# Autodesk Inventor assembly: Osnova
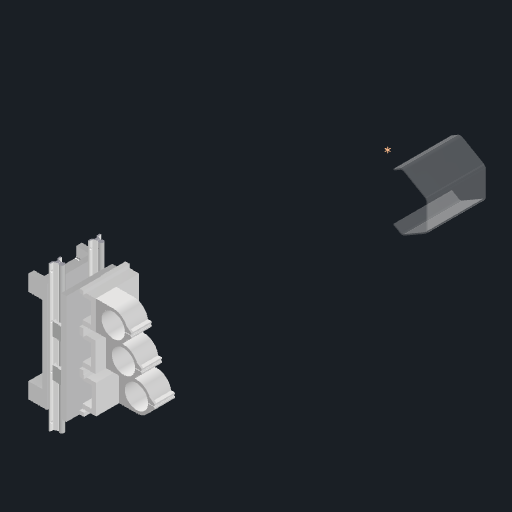
[picture p0: Inventor's stored thumbnail of the model, 512x512]
Saved by Autodesk Inventor 2024 (Build 280153000, 153)
## iProperties
Created: 2023-08-21
Part Number: Osnova
Document SubType Name: Assembly
Designer: KirikDK
Mass: 13525.1 g
Surface Area: 11415 cm^2
Volume: 6226.09 cm^3
Density: 2.17233 g/cm^3
Author: KirikDK
## Documents named in this file (8)
- C:\WorkProject\CNC_Lathe\MiniTocatka\BackSupport.iam
- C:\WorkProject\CNC_Lathe\MiniTocatka\Bear.ipt
- C:\WorkProject\CNC_Lathe\MiniTocatka\ZadBabkaOsnova.ipt
- C:\WorkProject\CNC_Lathe\MiniTocatka\PlasticZasita.ipt
- C:\WorkProject\CNC_Lathe\MiniTocatka\sbr16 (ap242)\0_8.ipt
- C:\WorkProject\CNC_Lathe\MiniTocatka\MotorClamp.ipt
- C:\WorkProject\CNC_Lathe\MiniTocatka\ZadBabkaPodkladka.ipt
- C:\WorkProject\CNC_Lathe\MiniTocatka\ZadBabkaBearsKrepl.ipt
## Components (15 placed, 7 different names)
1. ZadBabkaOsnova:2 — Mate:218, Mate:219, Flush:93, Flush:94
2. PlasticZasita:1
3. 0_8:1 — Mate:218, Flush:94, Mate:221, Mate:223
4. 0_8:2 — Mate:219, Flush:93, Mate:220, Mate:222
5. Bear:25 — Mate:223, Flush:96, Flush:98, Mate:229, Mate:237, Flush:108
6. Bear:26 — Mate:220, Flush:95, Flush:97
7. Bear:27 — Mate:221, Flush:95, Flush:97
8. Bear:28 — Mate:222, Flush:96, Flush:98
9. ZadBabkaPodkladka:1 — Mate:229, Mate:230, Flush:103, Mate:234, Flush:107, Mate:238, Flush:109
10. ZadBabkaPodkladka:2 — Mate:230, Flush:103, Flush:104, Mate:233, Mate:235, Flush:106
11. ZadBabkaPodkladka:3 — Flush:104, Mate:233, Mate:236, Flush:105
12. MotorClamp:3 — Mate:234, Flush:107
13. MotorClamp:4 — Mate:235, Flush:106
14. MotorClamp:5 — Mate:236, Flush:105
15. ZadBabkaBearsKrepl:1 — Mate:237, Flush:108, Mate:238, Flush:109
## Relationships (27: Mate 14, Flush 13)
- Mate:218: ZadBabkaOsnova:2 ↔ 0_8:1
- Mate:219: ZadBabkaOsnova:2 ↔ 0_8:2
- Flush:93: ZadBabkaOsnova:2 ↔ 0_8:2
- Flush:94: ZadBabkaOsnova:2 ↔ 0_8:1
- Mate:220: 0_8:2 ↔ Bear:26
- Mate:221: 0_8:1 ↔ Bear:27
- Mate:222: 0_8:2 ↔ Bear:28
- Mate:223: 0_8:1 ↔ Bear:25
- Flush:95: Bear:26 ↔ Bear:27
- Flush:96: Bear:25 ↔ Bear:28
- Flush:97: Bear:26 ↔ Bear:27
- Flush:98: Bear:25 ↔ Bear:28
- Mate:229: Bear:25 ↔ ZadBabkaPodkladka:1
- Mate:230: ZadBabkaPodkladka:1 ↔ ZadBabkaPodkladka:2
- Flush:103: ZadBabkaPodkladka:1 ↔ ZadBabkaPodkladka:2
- Flush:104: ZadBabkaPodkladka:2 ↔ ZadBabkaPodkladka:3
- Mate:233: ZadBabkaPodkladka:2 ↔ ZadBabkaPodkladka:3
- Mate:234: ZadBabkaPodkladka:1 ↔ MotorClamp:3
- Mate:235: ZadBabkaPodkladka:2 ↔ MotorClamp:4
- Mate:236: ZadBabkaPodkladka:3 ↔ MotorClamp:5
- Flush:105: ZadBabkaPodkladka:3 ↔ MotorClamp:5
- Flush:106: ZadBabkaPodkladka:2 ↔ MotorClamp:4
- Flush:107: ZadBabkaPodkladka:1 ↔ MotorClamp:3
- Mate:237: Bear:25 ↔ ZadBabkaBearsKrepl:1
- Flush:108: Bear:25 ↔ ZadBabkaBearsKrepl:1
- Mate:238: ZadBabkaPodkladka:1 ↔ ZadBabkaBearsKrepl:1
- Flush:109: ZadBabkaPodkladka:1 ↔ ZadBabkaBearsKrepl:1
